# Autodesk Inventor assembly: gripper2_v3
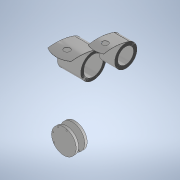
[picture p0: Inventor's stored thumbnail of the model, 180x180]
Saved by Autodesk Inventor 2022 (Build 260153000, 153)
## iProperties
Created: 2022-05-21
Part Number: gripper2_v3
Document SubType Name: Assembly
Designer: kylem
Author: kylem
## Documents named in this file (4)
- C:\Users\kylem\OneDrive\Documents\GitHub\IMML_Contactile_Gripper_Hardware\gripper_v2\gripper2_v3.iam
- C:\Users\kylem\OneDrive\Documents\GitHub\IMML_Contactile_Gripper_Hardware\gripper_v2\drum.ipt
- C:\Users\kylem\Downloads\9293K117_Constant-Force Spring.ipt
- C:\Users\kylem\Downloads\9293K263_Constant-Force Spring.ipt
## Components (4 placed, 3 different names)
1. drum:1 — Mate:3, Mate:4
2. drum:2 — Mate:1, Mate:2, Mate:3, Mate:4
3. 9293K117_Constant-Force Spring:1
4. 9293K263_Constant-Force Spring:1
## Relationships (4: Mate 4)
- Mate:1: drum:2
- Mate:2: drum:2
- Mate:3: drum:1 ↔ drum:2
- Mate:4 (5 mm): drum:1 ↔ drum:2
